# Autodesk Inventor assembly: Ensamble_Carcasa3.0
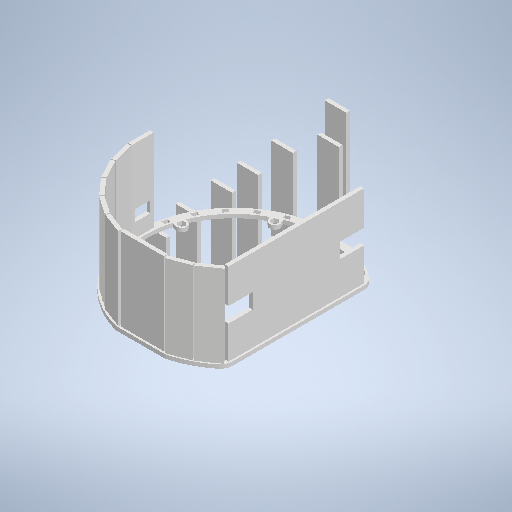
[picture p0: Inventor's stored thumbnail of the model, 512x512]
Saved by Autodesk Inventor 2025.3 (Build 293356030, 356C)
## iProperties
Created: 2025-09-09
Part Number: Ensamble_Carcasa3.0
Document SubType Name: Assembly
Designer: brene
Author: brene
## Documents named in this file (7)
- D:\OneDrive - Estudiantes ITCR\Documentos\GitHub\Atta-Bot-STEM\Chasis\Rediseño_Diego&Carlos\Piezas Carcasa 3.0\Ensamble_Carcasa3.0.iam
- D:\OneDrive - Estudiantes ITCR\Documentos\GitHub\Atta-Bot-STEM\Chasis\Rediseño_Diego&Carlos\Piezas Carcasa 3.0\carcasa3.0.ipt
- D:\OneDrive - Estudiantes ITCR\Documentos\GitHub\Atta-Bot-STEM\Chasis\Rediseño_Diego&Carlos\Piezas Carcasa 3.0\carcasa_piezaRadio_agujero_3.0.ipt
- D:\OneDrive - Estudiantes ITCR\Documentos\GitHub\Atta-Bot-STEM\Chasis\Rediseño_Diego&Carlos\Piezas Carcasa 3.0\carcasa_piezasRadio_3.0.ipt
- D:\OneDrive - Estudiantes ITCR\Documentos\GitHub\Atta-Bot-STEM\Chasis\Rediseño_Diego&Carlos\Piezas Carcasa 3.0\carcasa_piezaLateral_ruedas.ipt
- D:\OneDrive - Estudiantes ITCR\Documentos\GitHub\Atta-Bot-STEM\Chasis\Rediseño_Diego&Carlos\Piezas Carcasa 3.0\carcasa_piezaFrontal.ipt
- D:\OneDrive - Estudiantes ITCR\Documentos\GitHub\Atta-Bot-STEM\Chasis\Rediseño_Diego&Carlos\Piezas Carcasa 3.0\carcasa_piezaLateral_frontal.ipt
## Components (18 placed, 6 different names)
1. carcasa3.0:1 — Mate:1, Mate:2, Mate:3, Mate:4, Mate:5, Mate:6, Mate:7, Mate:8, Mate:9, Mate:10, Mate:11, Mate:12, Mate:13, Mate:14, Mate:15, Mate:16, Mate:17, Mate:18, Mate:19, Mate:20, Mate:21, Mate:22, Mate:23, Mate:24, Mate:25, Mate:26, Mate:27, Mate:28, Mate:29, Mate:30
2. carcasa_piezaRadio_agujero_3.0:1 — Mate:1, Mate:2, Mate:3
3. carcasa_piezasRadio_3.0:1 — Mate:4, Mate:5, Mate:6
4. carcasa_piezasRadio_3.0:2 — Mate:7, Mate:8, Mate:9
5. carcasa_piezasRadio_3.0:3 — Mate:10, Mate:11, Mate:12
6. carcasa_piezasRadio_3.0:4 — Mate:13, Mate:14, Mate:15
7. carcasa_piezasRadio_3.0:5 — Mate:16, Mate:17, Mate:18
8. carcasa_piezasRadio_3.0:6
9. carcasa_piezasRadio_3.0:7
10. carcasa_piezasRadio_3.0:8
11. carcasa_piezasRadio_3.0:9
12. carcasa_piezasRadio_3.0:10
13. carcasa_piezaLateral_ruedas:1 — Mate:19, Mate:20, Mate:21
14. carcasa_piezaFrontal:1 — Mate:22, Mate:23, Mate:24
15. carcasa_piezaLateral_frontal:1 — Mate:25, Mate:26, Mate:27
16. carcasa_piezaLateral_frontal:2 — Mate:28, Mate:29, Mate:30
17. carcasa_piezaLateral_frontal:3
18. carcasa_piezaLateral_frontal:4
## Relationships (30: Mate 30)
- Mate:1: carcasa3.0:1 ↔ carcasa_piezaRadio_agujero_3.0:1
- Mate:2: carcasa3.0:1 ↔ carcasa_piezaRadio_agujero_3.0:1
- Mate:3: carcasa3.0:1 ↔ carcasa_piezaRadio_agujero_3.0:1
- Mate:4: carcasa3.0:1 ↔ carcasa_piezasRadio_3.0:1
- Mate:5: carcasa3.0:1 ↔ carcasa_piezasRadio_3.0:1
- Mate:6: carcasa3.0:1 ↔ carcasa_piezasRadio_3.0:1
- Mate:7: carcasa3.0:1 ↔ carcasa_piezasRadio_3.0:2
- Mate:8: carcasa3.0:1 ↔ carcasa_piezasRadio_3.0:2
- Mate:9: carcasa3.0:1 ↔ carcasa_piezasRadio_3.0:2
- Mate:10: carcasa3.0:1 ↔ carcasa_piezasRadio_3.0:3
- Mate:11: carcasa3.0:1 ↔ carcasa_piezasRadio_3.0:3
- Mate:12: carcasa3.0:1 ↔ carcasa_piezasRadio_3.0:3
- Mate:13: carcasa3.0:1 ↔ carcasa_piezasRadio_3.0:4
- Mate:14: carcasa3.0:1 ↔ carcasa_piezasRadio_3.0:4
- Mate:15: carcasa3.0:1 ↔ carcasa_piezasRadio_3.0:4
- Mate:16: carcasa3.0:1 ↔ carcasa_piezasRadio_3.0:5
- Mate:17: carcasa3.0:1 ↔ carcasa_piezasRadio_3.0:5
- Mate:18: carcasa3.0:1 ↔ carcasa_piezasRadio_3.0:5
- Mate:19: carcasa3.0:1 ↔ carcasa_piezaLateral_ruedas:1
- Mate:20: carcasa3.0:1 ↔ carcasa_piezaLateral_ruedas:1
- Mate:21: carcasa3.0:1 ↔ carcasa_piezaLateral_ruedas:1
- Mate:22: carcasa3.0:1 ↔ carcasa_piezaFrontal:1
- Mate:23: carcasa3.0:1 ↔ carcasa_piezaFrontal:1
- Mate:24: carcasa3.0:1 ↔ carcasa_piezaFrontal:1
- Mate:25: carcasa3.0:1 ↔ carcasa_piezaLateral_frontal:1
- Mate:26: carcasa3.0:1 ↔ carcasa_piezaLateral_frontal:1
- Mate:27: carcasa3.0:1 ↔ carcasa_piezaLateral_frontal:1
- Mate:28: carcasa3.0:1 ↔ carcasa_piezaLateral_frontal:2
- Mate:29: carcasa3.0:1 ↔ carcasa_piezaLateral_frontal:2
- Mate:30: carcasa3.0:1 ↔ carcasa_piezaLateral_frontal:2
